# Autodesk Inventor assembly: FullTop
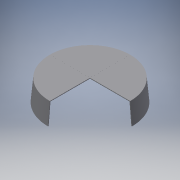
[picture p0: Inventor's stored thumbnail of the model, 180x180]
Saved by Autodesk Inventor 2019 (Build 230136000, 136)
## iProperties
Created: 2019-10-09
Part Number: FullTop
Document SubType Name: Assembly
Designer: james
Author: james
## Documents named in this file (2)
- F:\JimsDesign\Jims2020FTC\FullTop.iam
- F:\JimsDesign\Jims2020FTC\QuarterTop.ipt
## Components (3 placed, 1 different names)
1. QuarterTop:1 — Mate:1, Flush:1, Flush:2, Mate:2, Flush:3, Flush:4
2. QuarterTop:2 — Mate:2, Flush:3, Flush:4
3. QuarterTop:3 — Mate:1, Flush:1, Flush:2
## Relationships (6: Flush 4, Mate 2)
- Mate:1: QuarterTop:1 ↔ QuarterTop:3
- Flush:1: QuarterTop:1 ↔ QuarterTop:3
- Flush:2: QuarterTop:1 ↔ QuarterTop:3
- Mate:2: QuarterTop:1 ↔ QuarterTop:2
- Flush:3: QuarterTop:1 ↔ QuarterTop:2
- Flush:4: QuarterTop:1 ↔ QuarterTop:2
